# Autodesk Inventor assembly: fan_holder_0130
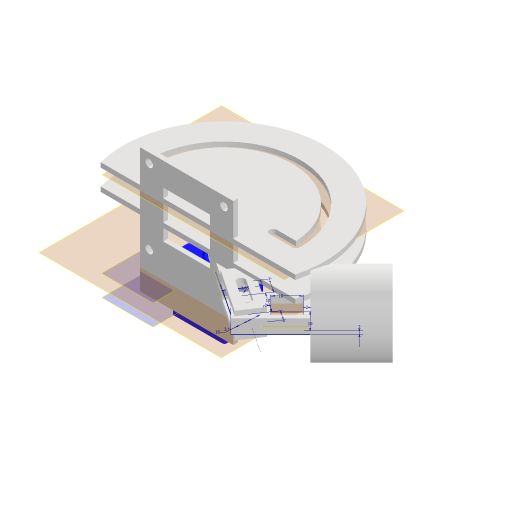
[picture p0: Inventor's stored thumbnail of the model, 512x512]
Saved by Autodesk Inventor 2024 (Build 280153000, 153)
## iProperties
Created: 2024-01-30
Part Number: fan_holder_0130
Document SubType Name: Assembly
Designer: admin
Author: admin
## Documents named in this file (7)
- C:\Users\admin\OneDrive\文件\碩士研究\prototype\fan_holder_0216\fan_holder_0216.iam
- C:\Users\admin\OneDrive\文件\碩士研究\prototype\fan_holder_0216\elemagnetic.ipt
- C:\Users\admin\OneDrive\文件\碩士研究\prototype\fan_holder_0216\elemagnetic_holder_0306.ipt
- C:\Users\admin\OneDrive\文件\碩士研究\prototype\fan_holder_0216\SG90 - Micro Servo 9g - Tower Pro.1_Pe_a.ipt
- C:\Users\admin\OneDrive\文件\碩士研究\prototype\fan_holder_0216\SG90 - Micro Servo 9g - Tower Pro.2_Pe_a.ipt
- C:\Users\admin\OneDrive\文件\碩士研究\prototype\fan_holder_0216\fan_holder_0301.ipt
- C:\Users\admin\OneDrive\文件\碩士研究\prototype\fan_holder_0216\SG90_holder_0213.ipt
## Components (6 placed, 6 different names)
1. elemagnetic:1 — 貼合:9, 貼合:10
2. elemagnetic_holder_0306:1 — 貼合:9, 貼合:10, 貼合:11, 貼合:12, 角度:1
3. SG90 - Micro Servo 9g - Tower Pro.1_Pe_a:1 — 貼合:1, 貼合:2, 貼合:3, 貼合:4, 貼合:5
4. SG90 - Micro Servo 9g - Tower Pro.2_Pe_a:1 — 貼合:4, 貼合:5, 貼合:6, 貼合:7, 貼合:8
5. fan_holder_0301:1 — 貼合:6, 貼合:7, 貼合:8, 貼合:11, 貼合:12
6. SG90_holder_0213:1 — 貼合:1, 貼合:2, 貼合:3, 角度:1
## Relationships (13: Mate 12, Angle 1)
- 貼合:1 [Mate]: SG90 - Micro Servo 9g - Tower Pro.1_Pe_a:1 ↔ SG90_holder_0213:1
- 貼合:2 [Mate]: SG90 - Micro Servo 9g - Tower Pro.1_Pe_a:1 ↔ SG90_holder_0213:1
- 貼合:3 [Mate]: SG90 - Micro Servo 9g - Tower Pro.1_Pe_a:1 ↔ SG90_holder_0213:1
- 貼合:4 [Mate]: SG90 - Micro Servo 9g - Tower Pro.1_Pe_a:1 ↔ SG90 - Micro Servo 9g - Tower Pro.2_Pe_a:1
- 貼合:5 [Mate]: SG90 - Micro Servo 9g - Tower Pro.1_Pe_a:1 ↔ SG90 - Micro Servo 9g - Tower Pro.2_Pe_a:1
- 貼合:6 [Mate]: SG90 - Micro Servo 9g - Tower Pro.2_Pe_a:1 ↔ fan_holder_0301:1
- 貼合:7 [Mate]: SG90 - Micro Servo 9g - Tower Pro.2_Pe_a:1 ↔ fan_holder_0301:1
- 貼合:8 [Mate]: SG90 - Micro Servo 9g - Tower Pro.2_Pe_a:1 ↔ fan_holder_0301:1
- 貼合:9 [Mate]: elemagnetic:1 ↔ elemagnetic_holder_0306:1
- 貼合:10 [Mate]: elemagnetic:1 ↔ elemagnetic_holder_0306:1
- 貼合:11 [Mate]: elemagnetic_holder_0306:1 ↔ fan_holder_0301:1
- 貼合:12 [Mate]: elemagnetic_holder_0306:1 ↔ fan_holder_0301:1
- 角度:1 [Angle] (135 deg): elemagnetic_holder_0306:1 ↔ SG90_holder_0213:1
